# Autodesk Inventor assembly: Board
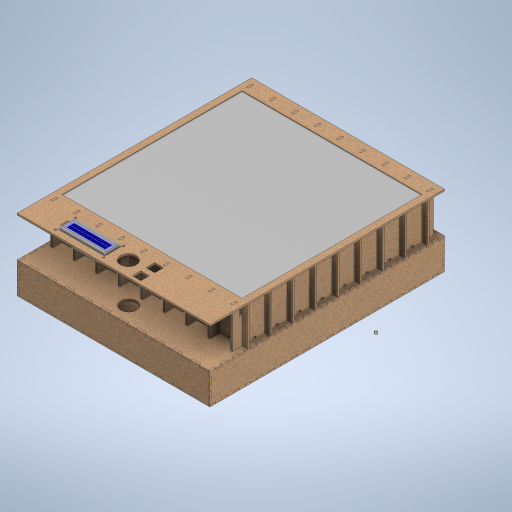
[picture p0: Inventor's stored thumbnail of the model, 512x512]
Saved by Autodesk Inventor 2024 (Build 280153000, 153)
## iProperties
Created: 2023-07-19
Part Number: Board
Document SubType Name: Assembly
Designer: Bruno
Author: Bruno
## Documents named in this file (10)
- C:\Users\Bruno\brucloud\utn\td2\proyecto\autodesk\MagicChess.iam
- C:\Users\Bruno\brucloud\utn\td2\proyecto\autodesk\TopBoard.ipt
- C:\Users\Bruno\brucloud\utn\td2\proyecto\autodesk\SeparatorAssembly.iam
- C:\Users\Bruno\brucloud\utn\td2\proyecto\autodesk\LedBoard.ipt
- C:\Users\Bruno\brucloud\utn\td2\proyecto\autodesk\1602-lcd-display-1.snapshot.2\1602 Serial LCD Module Display\1602 Serial LCD Module Display.ipt
- C:\Users\Bruno\brucloud\utn\td2\proyecto\autodesk\BaseBoard.ipt
- C:\Users\Bruno\brucloud\utn\td2\proyecto\autodesk\SideWall.ipt
- C:\Users\Bruno\brucloud\utn\td2\proyecto\autodesk\BackWall.ipt
- C:\Users\Bruno\brucloud\utn\td2\proyecto\autodesk\FrontWall.ipt
- C:\Users\Bruno\brucloud\utn\td2\proyecto\autodesk\Window.ipt
## Components (10 placed, 9 different names)
1. TopBoard:1 — Rigid:2, Cylindrical:1, Angle:1, Mate:1, Flush:1, Flush:2
2. SeparatorAssembly:1 [sub-assembly] — Rigid:2, Flush:3, Flush:15
3. LedBoard:1 — Flush:1, Flush:2, Flush:3, Flush:7
4. 1602 Serial LCD Module Display:1 — Cylindrical:1, Angle:1, Mate:1
5. BaseBoard:1 — Flush:4, Flush:5, Flush:6, Flush:8, Flush:9, Flush:10
6. SideWall:1 — Flush:4, Flush:5, Flush:6, Flush:7, Mate:2
7. SideWall:2 — Flush:8, Flush:9, Flush:10, Flush:11
8. FrontWall:1 — Mate:2
9. BackWall:1 — Flush:11
10. Window:1 — Flush:15
## Relationships (19: Flush 14, Mate 2, WeldJoint 1, CylindricalJoint 1, Angle 1)
- Rigid:2 [WeldJoint]: TopBoard:1 ↔ SeparatorAssembly:1
- Cylindrical:1: TopBoard:1 ↔ 1602 Serial LCD Module Display:1
- Angle:1 (0 deg): TopBoard:1 ↔ 1602 Serial LCD Module Display:1
- Mate:1: TopBoard:1 ↔ 1602 Serial LCD Module Display:1
- Flush:1: TopBoard:1 ↔ LedBoard:1
- Flush:2: TopBoard:1 ↔ LedBoard:1
- Flush:3: SeparatorAssembly:1 ↔ LedBoard:1
- Flush:4: BaseBoard:1 ↔ SideWall:1
- Flush:5: BaseBoard:1 ↔ SideWall:1
- Flush:6: BaseBoard:1 ↔ SideWall:1
- Flush:7: LedBoard:1 ↔ SideWall:1
- Flush:8: BaseBoard:1 ↔ SideWall:2
- Flush:9: BaseBoard:1 ↔ SideWall:2
- Flush:10: BaseBoard:1 ↔ SideWall:2
- Flush:11: SideWall:2 ↔ BackWall:1
- [Flush]: BaseBoard:1 ↔ FrontWall:1
- [Flush]: BaseBoard:1 ↔ FrontWall:1
- Mate:2: SideWall:1 ↔ FrontWall:1
- Flush:15: SeparatorAssembly:1 ↔ Window:1
